# Autodesk Inventor assembly: Table_ajutable_part
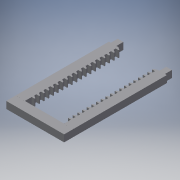
[picture p0: Inventor's stored thumbnail of the model, 180x180]
Saved by Autodesk Inventor 2019.4 (Build 234330000, 330)
## iProperties
Created: 2019-12-14
Part Number: Table_ajutable_part
Document SubType Name: Assembly
Designer: fabfarm
Author: fabfarm
## Documents named in this file (3)
- D:\Users\fabfarm\Documents\Saw table\Table_ajutable_part.iam
- D:\Users\fabfarm\Documents\Saw table\mobile_table_bottom.ipt
- D:\Users\fabfarm\Documents\Saw table\graduated_foot.ipt
## Components (6 placed, 2 different names)
1. mobile_table_bottom:1 — Flush:1, Mate:1, Mate:2, Flush:3, Flush:4, Flush:5, Mate:6, Flush:10
2. graduated_foot:1 — Flush:1, Mate:1, Flush:3, Flush:6, Mate:3, Flush:7
3. graduated_foot:2 — Mate:2, Flush:4, Flush:5, Mate:4, Flush:8, Flush:9
4. graduated_foot:3 — Flush:6, Mate:3, Flush:7, Mate:5
5. graduated_foot:4 — Mate:4, Flush:8, Flush:9
6. mobile_table_bottom:2 — Mate:5, Mate:6, Flush:10
## Relationships (15: Flush 9, Mate 6)
- Flush:1: mobile_table_bottom:1 ↔ graduated_foot:1
- Mate:1: mobile_table_bottom:1 ↔ graduated_foot:1
- Mate:2: mobile_table_bottom:1 ↔ graduated_foot:2
- Flush:3: mobile_table_bottom:1 ↔ graduated_foot:1
- Flush:4: mobile_table_bottom:1 ↔ graduated_foot:2
- Flush:5: mobile_table_bottom:1 ↔ graduated_foot:2
- Flush:6: graduated_foot:1 ↔ graduated_foot:3
- Mate:3: graduated_foot:1 ↔ graduated_foot:3
- Flush:7: graduated_foot:1 ↔ graduated_foot:3
- Mate:4: graduated_foot:2 ↔ graduated_foot:4
- Flush:8: graduated_foot:2 ↔ graduated_foot:4
- Flush:9: graduated_foot:2 ↔ graduated_foot:4
- Mate:5: graduated_foot:3 ↔ mobile_table_bottom:2
- Mate:6: mobile_table_bottom:1 ↔ mobile_table_bottom:2
- Flush:10: mobile_table_bottom:1 ↔ mobile_table_bottom:2
